# Autodesk Inventor assembly: Frame
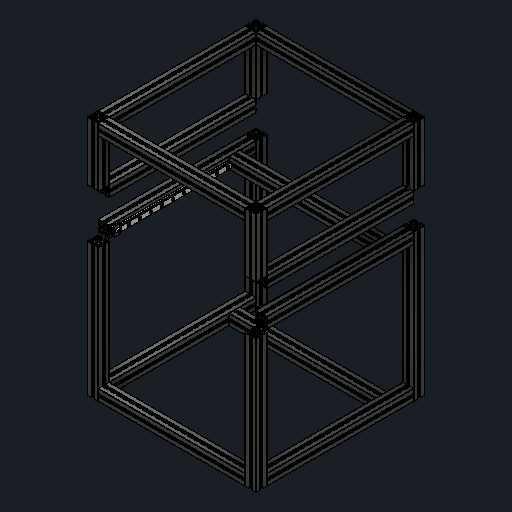
[picture p0: Inventor's stored thumbnail of the model, 512x512]
Saved by Autodesk Inventor 2026.2 (Build 302298000, 298)
## iProperties
Created: 2025-05-09
Part Number: Frame
Document SubType Name: Assembly
Designer: AdminForWorker
Title: Frame
Author: AdminForWorker
## Documents named in this file (13)
- C:\Users\JoshuaEah\Documents\GitHub\Voron-0\CAD\Frame\Frame.iam
- C:\Users\JoshuaEah\Documents\GitHub\Voron-0\CAD\Hardware\Linear Rail\MGN7 Rail 150mm.iam
- MGN7 150mm Rail.iam
- C:\Users\JoshuaEah\Documents\GitHub\Voron-0\CAD\Frame\Parts\Rail Stop.iam
- C:\Users\JoshuaEah\Documents\GitHub\Voron-0\CAD\Frame\Foam Tape.iam
- C:\Users\JoshuaEah\Documents\GitHub\Voron-0\CAD\Frame\Parts\1515_200mm - E.ipt
- C:\Users\JoshuaEah\Documents\GitHub\Voron-0\CAD\Frame\Parts\1515_200mm - C.ipt
- C:\Users\JoshuaEah\Documents\GitHub\Voron-0\CAD\Frame\Parts\1515_200mm - B.ipt
- C:\Users\JoshuaEah\Documents\GitHub\Voron-0\CAD\Hardware\Fasteners\M3x8 BHCS.ipt
- C:\Users\JoshuaEah\Documents\GitHub\Voron-0\CAD\Hardware\Fasteners\M3x10 BHCS.ipt
- C:\Users\JoshuaEah\Documents\GitHub\Voron-0\CAD\Frame\Parts\1515 200mm - A.ipt
- C:\Users\JoshuaEah\Documents\GitHub\Voron-0\CAD\Frame\Parts\1515 80mm - H.ipt
- C:\Users\JoshuaEah\Documents\GitHub\Voron-0\CAD\Frame\Parts\1515_200mm - D (Alternate).ipt
## Components (48 placed, 11 different names)
1. MGN7 150mm Rail:3 [sub-assembly] — Mate:20
2. MGN7 150mm Rail:4 [sub-assembly] — Mate:22
3. Rail Stop:1 [sub-assembly] — Mate:20
4. Rail Stop:2 [sub-assembly] — Mate:22
5. Foam Tape:1 [sub-assembly]
6. 1515 200mm - A:1
7. 1515 200mm - A:2
8. 1515 200mm - A:3
9. 1515 200mm - A:4
10. 1515_200mm - C:1
11. 1515_200mm - C:2
12. 1515_200mm - B:1 — Flush:115, Flush:116
13. 1515_200mm - B:2
14. 1515_200mm - B:3
15. 1515_200mm - B:4
16. 1515_200mm - B:5
17. 1515_200mm - D:1 — Flush:116
18. 1515_200mm - D:2 — Flush:115
19. 1515_200mm - E:1
20. 1515_200mm - E:2
21. 1515_200mm - E:3
22. 1515_200mm - E:4
23. 1515 80mm - H:1
24. 1515 80mm - H:2
25. 1515 80mm - H:3
26. 1515 80mm - H:4
27. M3x8 BHCS:1
28. M3x8 BHCS:2
29. M3x8 BHCS:3
30. M3x8 BHCS:4
31. M3x8 BHCS:5
32. M3x8 BHCS:6
33. M3x8 BHCS:7
34. M3x8 BHCS:8
35. M3x8 BHCS:9
36. M3x8 BHCS:11
37. M3x8 BHCS:13
38. M3x8 BHCS:14
39. M3x8 BHCS:35
40. M3x8 BHCS:36
41. M3x10 BHCS:1
42. M3x10 BHCS:2
43. M3x10 BHCS:3
44. M3x10 BHCS:4
45. M3x10 BHCS:5
46. M3x10 BHCS:6
47. M3x10 BHCS:7
48. M3x10 BHCS:8
## Relationships (148: Mate 77, Flush 71)
- [Mate]: MGN7 150mm Rail:3 ↔ 1515_200mm - E:1
- [Mate] (0.1 mm): MGN7 150mm Rail:3 ↔ 1515_200mm - E:1
- [Flush] (38 mm): MGN7 150mm Rail:3 ↔ 1515_200mm - E:1
- [Flush] (38 mm): MGN7 150mm Rail:4 ↔ 1515_200mm - E:3
- [Mate]: MGN7 150mm Rail:4 ↔ 1515_200mm - E:3
- [Mate] (0.1 mm): MGN7 150mm Rail:4 ↔ 1515_200mm - E:3
- [Mate]: Rail Stop:1 ↔ 1515_200mm - E:1
- Mate:20: MGN7 150mm Rail:3 ↔ Rail Stop:1
- [Flush]: Rail Stop:1 ↔ 1515_200mm - E:1
- [Mate]: Rail Stop:2 ↔ 1515_200mm - E:3
- Mate:22: MGN7 150mm Rail:4 ↔ Rail Stop:2
- [Flush]: Rail Stop:2 ↔ 1515_200mm - E:3
- [Mate]: Foam Tape:1 ↔ 1515_200mm - E:1
- [Flush]: Foam Tape:1 ↔ 1515_200mm - E:1
- [Mate]: Foam Tape:1 ↔ 1515_200mm - E:4
- [Flush]: Foam Tape:1 ↔ 1515_200mm - E:4
- [Mate]: Foam Tape:1 ↔ 1515_200mm - E:3
- [Flush]: Foam Tape:1 ↔ 1515_200mm - E:3
- [Mate]: Foam Tape:1 ↔ 1515_200mm - E:2
- [Flush]: Foam Tape:1 ↔ 1515_200mm - E:2
- [Mate]: Foam Tape:1 ↔ 1515 200mm - A:1
- [Flush]: Foam Tape:1 ↔ 1515 200mm - A:1
- [Flush]: Foam Tape:1 ↔ 1515 200mm - A:1
- [Mate]: Foam Tape:1 ↔ 1515_200mm - B:3
- [Flush]: Foam Tape:1 ↔ 1515_200mm - B:3
- [Flush]: Foam Tape:1 ↔ 1515_200mm - B:3
- [Mate]: Foam Tape:1 ↔ 1515 200mm - A:3
- [Flush]: Foam Tape:1 ↔ 1515 200mm - A:3
- [Flush]: Foam Tape:1 ↔ 1515 200mm - A:3
- [Mate]: Foam Tape:1 ↔ 1515_200mm - B:2
- [Flush]: Foam Tape:1 ↔ 1515_200mm - B:2
- [Flush]: Foam Tape:1 ↔ 1515_200mm - B:2
- [Mate]: Foam Tape:1 ↔ 1515 80mm - H:1
- [Flush]: Foam Tape:1 ↔ 1515 80mm - H:1
- [Flush]: Foam Tape:1 ↔ 1515 80mm - H:1
- [Mate]: Foam Tape:1 ↔ 1515 80mm - H:3
- [Flush]: Foam Tape:1 ↔ 1515 80mm - H:3
- [Flush]: Foam Tape:1 ↔ 1515 80mm - H:3
- [Mate]: Foam Tape:1 ↔ 1515_200mm - C:2
- [Flush]: Foam Tape:1 ↔ 1515_200mm - C:2
- [Flush]: Foam Tape:1 ↔ 1515_200mm - C:2
- [Mate]: Foam Tape:1 ↔ 1515_200mm - D:2
- [Flush]: Foam Tape:1 ↔ 1515_200mm - D:2
- [Flush]: Foam Tape:1 ↔ 1515_200mm - E:4
- [Flush]: Foam Tape:1 ↔ 1515_200mm - E:1
- [Mate]: Foam Tape:1 ↔ 1515_200mm - D:1
- [Flush]: Foam Tape:1 ↔ 1515_200mm - D:1
- [Mate]: Foam Tape:1 ↔ 1515_200mm - C:1
- [Flush]: Foam Tape:1 ↔ 1515_200mm - C:1
- [Flush]: Foam Tape:1 ↔ 1515_200mm - C:1
- [Flush]: Foam Tape:1 ↔ 1515_200mm - E:2
- [Flush]: Foam Tape:1 ↔ 1515_200mm - E:3
- [Mate]: Foam Tape:1 ↔ 1515 80mm - H:4
- [Flush]: Foam Tape:1 ↔ 1515 80mm - H:4
- [Flush]: Foam Tape:1 ↔ 1515 80mm - H:4
- [Mate]: Foam Tape:1 ↔ 1515 80mm - H:2
- [Flush]: Foam Tape:1 ↔ 1515 80mm - H:2
- [Flush]: Foam Tape:1 ↔ 1515 80mm - H:2
- [Mate]: Foam Tape:1 ↔ 1515_200mm - D:2
- [Flush]: Foam Tape:1 ↔ 1515_200mm - D:2
- [Mate]: Foam Tape:1 ↔ 1515_200mm - D:1
- [Flush]: Foam Tape:1 ↔ 1515_200mm - D:1
- [Mate]: Foam Tape:1 ↔ 1515 80mm - H:4
- [Flush]: Foam Tape:1 ↔ 1515 80mm - H:4
- [Flush]: Foam Tape:1 ↔ 1515 80mm - H:4
- [Mate]: Foam Tape:1 ↔ 1515 80mm - H:3
- [Flush]: Foam Tape:1 ↔ 1515 80mm - H:3
- [Flush]: Foam Tape:1 ↔ 1515 80mm - H:3
- [Mate]: Foam Tape:1 ↔ 1515_200mm - B:1
- [Flush]: Foam Tape:1 ↔ 1515_200mm - B:1
- [Flush]: Foam Tape:1 ↔ 1515_200mm - B:1
- [Mate]: Foam Tape:1 ↔ 1515 200mm - A:4
- [Flush]: Foam Tape:1 ↔ 1515 200mm - A:4
- [Flush]: Foam Tape:1 ↔ 1515 200mm - A:4
- [Mate]: Foam Tape:1 ↔ 1515 200mm - A:1
- [Flush]: Foam Tape:1 ↔ 1515 200mm - A:1
- [Flush]: Foam Tape:1 ↔ 1515 200mm - A:1
- [Mate]: Foam Tape:1 ↔ 1515 200mm - A:3
- [Flush]: Foam Tape:1 ↔ 1515 200mm - A:3
- [Flush]: Foam Tape:1 ↔ 1515 200mm - A:3
- [Mate]: Foam Tape:1 ↔ 1515_200mm - C:1
- [Flush]: Foam Tape:1 ↔ 1515_200mm - C:1
- [Flush]: Foam Tape:1 ↔ 1515_200mm - C:1
- [Mate]: Foam Tape:1 ↔ 1515_200mm - C:2
- [Flush]: Foam Tape:1 ↔ 1515_200mm - C:2
- [Flush]: Foam Tape:1 ↔ 1515_200mm - C:2
- [Mate]: Foam Tape:1 ↔ 1515 80mm - H:2
- [Flush]: Foam Tape:1 ↔ 1515 80mm - H:2
- [Flush]: Foam Tape:1 ↔ 1515 80mm - H:2
- [Mate]: Foam Tape:1 ↔ 1515 80mm - H:1
- [Flush]: Foam Tape:1 ↔ 1515 80mm - H:1
- [Flush]: Foam Tape:1 ↔ 1515 80mm - H:1
- [Mate]: Foam Tape:1 ↔ 1515 200mm - A:2
- [Flush]: Foam Tape:1 ↔ 1515 200mm - A:2
- [Flush]: Foam Tape:1 ↔ 1515 200mm - A:2
- [Flush]: 1515_200mm - D:2 ↔ 1515_200mm - E:1
- [Mate]: 1515_200mm - D:2 ↔ 1515_200mm - E:1
- [Mate]: 1515_200mm - C:2 ↔ M3x8 BHCS:11
- [Mate]: 1515_200mm - C:2 ↔ M3x8 BHCS:11
- [Mate]: 1515_200mm - C:1 ↔ M3x8 BHCS:9
- [Mate]: 1515_200mm - C:1 ↔ M3x8 BHCS:9
- [Mate]: 1515_200mm - E:4 ↔ M3x8 BHCS:7
- [Mate]: 1515_200mm - E:4 ↔ M3x8 BHCS:3
- [Mate]: 1515_200mm - E:2 ↔ M3x8 BHCS:4
- [Mate]: 1515_200mm - E:2 ↔ M3x8 BHCS:8
- [Mate]: 1515_200mm - C:2 ↔ M3x8 BHCS:7
- [Mate]: 1515_200mm - C:2 ↔ 1515_200mm - E:4
- [Flush]: 1515_200mm - C:2 ↔ 1515_200mm - E:4
- [Flush]: 1515_200mm - C:2 ↔ 1515_200mm - E:4
- [Mate]: 1515_200mm - D:2 ↔ M3x8 BHCS:3
- [Mate]: 1515_200mm - D:2 ↔ 1515_200mm - E:4
- [Flush]: 1515_200mm - D:2 ↔ 1515_200mm - E:4
- [Mate]: 1515_200mm - B:1 ↔ M3x8 BHCS:5
- [Mate]: 1515_200mm - B:1 ↔ M3x8 BHCS:2
- [Mate]: 1515_200mm - D:2 ↔ M3x8 BHCS:2
- [Mate]: 1515_200mm - D:1 ↔ M3x8 BHCS:5
- [Flush]: 1515_200mm - B:1 ↔ 1515_200mm - D:1
- [Mate]: 1515_200mm - B:1 ↔ 1515_200mm - D:1
- [Mate]: 1515_200mm - B:1 ↔ 1515_200mm - D:2
- [Flush]: 1515_200mm - B:1 ↔ 1515_200mm - D:2
- [Mate]: 1515_200mm - E:3 ↔ M3x8 BHCS:9
- [Mate]: 1515_200mm - C:1 ↔ 1515_200mm - E:3
- [Mate]: 1515_200mm - D:1 ↔ 1515_200mm - E:3
- [Flush]: 1515_200mm - D:1 ↔ 1515_200mm - E:2
- [Mate]: 1515_200mm - C:1 ↔ M3x8 BHCS:8
- [Mate]: 1515_200mm - D:1 ↔ M3x8 BHCS:4
- [Mate]: 1515_200mm - D:1 ↔ 1515_200mm - E:2
- [Mate]: 1515_200mm - B:4 ↔ M3x8 BHCS:6
- [Mate]: 1515_200mm - B:4 ↔ M3x8 BHCS:1
- [Mate]: 1515_200mm - E:2 ↔ M3x8 BHCS:6
- [Mate]: 1515_200mm - E:4 ↔ M3x8 BHCS:1
- [Mate]: 1515_200mm - B:4 ↔ 1515_200mm - E:4
- [Mate]: 1515_200mm - E:4 ↔ M3x8 BHCS:1
- [Mate]: 1515_200mm - E:2 ↔ M3x8 BHCS:6
- [Flush]: 1515_200mm - B:4 ↔ 1515_200mm - E:4
- [Mate]: 1515_200mm - B:5 ↔ M3x8 BHCS:13
- [Mate]: 1515_200mm - B:5 ↔ M3x8 BHCS:14
- [Mate]: 1515_200mm - E:1 ↔ M3x8 BHCS:14
- [Flush]: 1515_200mm - C:1 ↔ 1515_200mm - E:3
- [Mate]: 1515_200mm - E:3 ↔ M3x8 BHCS:13
- [Mate]: 1515_200mm - E:3 ↔ M3x8 BHCS:13
- [Mate]: 1515_200mm - E:1 ↔ M3x8 BHCS:14
- [Flush]: 1515_200mm - B:5 ↔ 1515_200mm - E:3
- [Mate]: 1515_200mm - B:5 ↔ 1515_200mm - E:3
- [Flush]: 1515_200mm - B:2 ↔ 1515 80mm - H:4
- [Mate]: 1515_200mm - B:2 ↔ 1515 80mm - H:4
- Flush:115: 1515_200mm - B:1 ↔ 1515_200mm - D:2
- Flush:116: 1515_200mm - B:1 ↔ 1515_200mm - D:1
## Named parameters: d167_d49 = 0 mm, d168_d50 = 0 mm, d179_d61 = 0 mm, d180_d62 = 0 mm, d182_d64 = 0 mm, d183_d65 = 0 mm, d185_d67 = 0 mm, d186_d68 = 0 mm, d187_d69 = 0 mm, d188_d70 = 0 mm, d189_d71 = 0 mm, d190_d77 = 0 mm, d191_d78 = 0 mm, d205_d25 = 0 mm, d206_d26 = 0 mm, d207_d27 = 0 mm, d208_d28 = 0 mm, d209_d29 = 0 mm, d210_d30 = 0 mm, d218_d38 = 0 mm, d219_d39 = 0 mm, d220_d40 = 0 mm, d222_d42 = 0 mm
